# Autodesk Inventor assembly: main room with double door
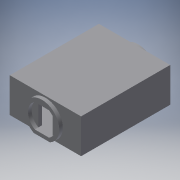
[picture p0: Inventor's stored thumbnail of the model, 180x180]
Saved by Autodesk Inventor 2017 (Build 210142000, 142)
## iProperties
Created: 2018-03-03
Part Number: main room with double door
Document SubType Name: Assembly
Designer: Braxton
Author: Braxton
## Documents named in this file (3)
- E:\School\Game develpment\geoscape\done\rooms\assembly\main room with double door.iam
- E:\School\Game develpment\geoscape\done\rooms\starting room.ipt
- E:\School\Game develpment\geoscape\done\doors\double door.ipt
## Components (3 placed, 3 different names)
1. starting room:1 — Mate:1, Mate:2, Flush:1, Mate:3, Mate:4, Flush:2
2. right double door:1 — Mate:1, Mate:2, Flush:1
3. left double door:2 — Mate:3, Mate:4, Flush:2
## Relationships (6: Mate 4, Flush 2)
- Mate:1: starting room:1 ↔ right double door:1
- Mate:2: starting room:1 ↔ right double door:1
- Flush:1: starting room:1 ↔ right double door:1
- Mate:3: starting room:1 ↔ left double door:2
- Mate:4: starting room:1 ↔ left double door:2
- Flush:2: starting room:1 ↔ left double door:2
